# Autodesk Inventor assembly: 組合1
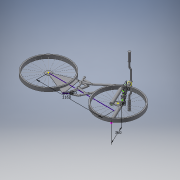
[picture p0: Inventor's stored thumbnail of the model, 180x180]
Saved by Autodesk Inventor 2019 (Build 230136000, 136)
## iProperties
Created: 2021-03-25
Part Number: 組合1
Material: 一般
Document SubType Name: Assembly
Designer: cadlab
Author: cadlab
## Documents named in this file (10)
- F:\pyslvs.io\project3\40723102\bick\組合1.iam
- F:\pyslvs.io\project3\40723102\bick\bick1.ipt
- F:\pyslvs.io\project3\40723102\bick\test.ipt
- F:\pyslvs.io\project3\40723102\bick\test3.ipt
- F:\pyslvs.io\project3\40723102\bick\test6.ipt
- F:\pyslvs.io\project3\40723102\bick\圓柱.ipt
- F:\pyslvs.io\project3\40723102\bick\圓柱3.ipt
- F:\pyslvs.io\project3\40723102\bick\前桿2.ipt
- F:\pyslvs.io\project3\40723102\bick\方向桿.ipt
- F:\pyslvs.io\project3\40723102\bick\輪子.ipt
## Components (10 placed, 9 different names)
1. bick1:1 — 貼合:7, 齊平:2, 貼合:8, 貼合:10, 圓柱:2
2. test:1 — 貼合:3, 貼合:5, 齊平:2, 角度:1, 貼合:11, 齊平:7
3. test6:2 — 貼合:3, 齊平:4, 貼合:8
4. test3:1 — 貼合:5, 齊平:1, 貼合:7, 貼合:9
5. 圓柱:1 — 貼合:9, 齊平:5, 圓柱:1
6. 圓柱3:1 — 齊平:6, 圓柱:1, 貼合:10
7. 前桿2:1 — 圓柱:2, 角度:1, 貼合:12, 插入:1
8. 輪子:1 — 貼合:11, 齊平:7
9. 輪子:2 — 貼合:12
10. 方向桿:1 — 插入:1
## Relationships (18: Mate 8, Flush 6, CylindricalJoint 2, Angle 1, Insert 1)
- 貼合:3 [Mate]: test:1 ↔ test6:2
- 貼合:5 [Mate]: test:1 ↔ test3:1
- 齊平:1 [Flush]: test3:1
- 貼合:7 [Mate]: bick1:1 ↔ test3:1
- 齊平:2 [Flush]: bick1:1 ↔ test:1
- 齊平:4 [Flush]: test6:2
- 貼合:8 [Mate]: bick1:1 ↔ test6:2
- 貼合:9 [Mate]: test3:1 ↔ 圓柱:1
- 齊平:5 [Flush]: 圓柱:1
- 齊平:6 [Flush]: 圓柱3:1
- 圓柱:1 [CylindricalJoint]: 圓柱:1 ↔ 圓柱3:1
- 貼合:10 [Mate]: bick1:1 ↔ 圓柱3:1
- 圓柱:2 [CylindricalJoint]: bick1:1 ↔ 前桿2:1
- 角度:1 [Angle] (0 deg): test:1 ↔ 前桿2:1
- 貼合:11 [Mate]: test:1 ↔ 輪子:1
- 齊平:7 [Flush]: test:1 ↔ 輪子:1
- 貼合:12 [Mate]: 前桿2:1 ↔ 輪子:2
- 插入:1 [Insert]: 前桿2:1 ↔ 方向桿:1
